# Autodesk Inventor assembly: parte_superior
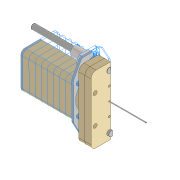
[picture p0: Inventor's stored thumbnail of the model, 180x180]
Saved by Autodesk Inventor 2020 (Build 240168000, 168)
## iProperties
Created: 2022-07-16
Part Number: parte_superior
Document SubType Name: Assembly
Designer: gabri
Author: gabri
## Documents named in this file (6)
- C:\Users\gabri\OneDrive\Área de Trabalho\Calorimetro 2022\Inventor\parte_superior.iam
- C:\Users\gabri\OneDrive\Área de Trabalho\Calorimetro 2022\Inventor\termopar.ipt
- C:\Users\gabri\OneDrive\Área de Trabalho\Calorimetro 2022\Inventor\Inferior_base.ipt
- C:\Users\gabri\OneDrive\Área de Trabalho\Calorimetro 2022\Inventor\Montagem_corpo_menor.iam
- C:\Users\gabri\OneDrive\Área de Trabalho\Calorimetro 2022\Inventor\guia_10mm.ipt
- C:\Users\gabri\OneDrive\Área de Trabalho\Calorimetro 2022\Inventor\Inferior_encaixe.ipt
## Components (7 placed, 5 different names)
1. termopar:1 — Coincidência:10, Coincidência:17
2. Montagem_corpo_menor:1 [sub-assembly] — Coincidência:13
3. guia_10mm:1 — Coincidência:11
4. guia_10mm:2 — Coincidência:12, Coincidência:13
5. Inferior_encaixe:1 — Coincidência:15, Coincidência:16, Coincidência:17
6. Inferior_base:1 — Coincidência:10, Coincidência:11, Coincidência:12, Coincidência:15, Coincidência:16
7. Inferior_base:2
## Component patterns: (2 elements, first: Inferior_base:1)
## Relationships (7: Mate 7)
- Coincidência:10 [Mate]: termopar:1 ↔ Inferior_base:1
- Coincidência:11 [Mate]: guia_10mm:1 ↔ Inferior_base:1
- Coincidência:12 [Mate]: guia_10mm:2 ↔ Inferior_base:1
- Coincidência:13 [Mate]: Montagem_corpo_menor:1 ↔ guia_10mm:2
- Coincidência:15 [Mate]: Inferior_encaixe:1 ↔ Inferior_base:1
- Coincidência:16 [Mate]: Inferior_encaixe:1 ↔ Inferior_base:1
- Coincidência:17 [Mate]: termopar:1 ↔ Inferior_encaixe:1
